# Autodesk Inventor assembly: Boost Converter
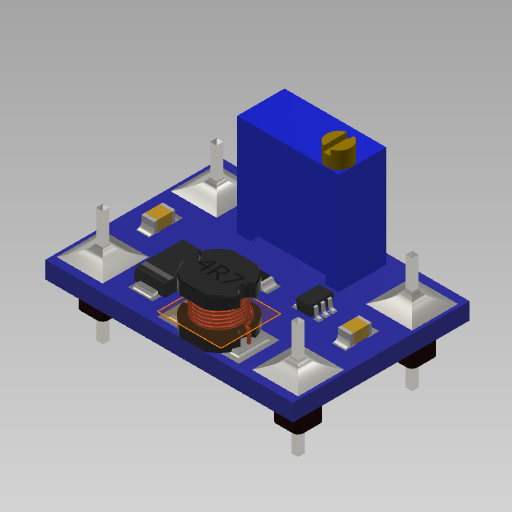
[picture p0: Inventor's stored thumbnail of the model, 512x512]
Saved by Autodesk Inventor 2020 (Build 240168000, 168)
## iProperties
Created: 2018-09-30
Part Number: Boost Converter
Document SubType Name: Weldment
Designer: amsmi
Weld Material: Titanium
Author: amsmi
## Documents named in this file (9)
- C:\Users\Alex\Google Drive\Pirani Gauge\Pirani Gauge Modeling\Data Acquisition\Boost Converter.iam
- C:\Users\Alex\Google Drive\Pirani Gauge\Pirani Gauge Modeling\Data Acquisition\Boost Converter.ipt
- C:\Users\Alex\Google Drive\Pirani Gauge\Pirani Gauge Modeling\Data Acquisition\DO-221AC.ipt
- C:\Users\Alex\Google Drive\Pirani Gauge\Pirani Gauge Modeling\Data Acquisition\Cap 0805.ipt
- C:\Users\Alex\Google Drive\Pirani Gauge\Pirani Gauge Modeling\Data Acquisition\Precision Trim Pot - baoter 3296.ipt
- C:\Users\Alex\Google Drive\Pirani Gauge\Pirani Gauge Modeling\Data Acquisition\Black 0805.ipt
- C:\Users\Alex\Google Drive\Pirani Gauge\Pirani Gauge Modeling\Data Acquisition\400nH Inductor.ipt
- C:\Users\Alex\Google Drive\Pirani Gauge\Pirani Gauge Modeling\Data Acquisition\SOT-23 6 pin.iam
- C:\Users\Alex\Google Drive\Pirani Gauge\Pirani Gauge Modeling\Data Acquisition\1 pin header.ipt
## Components (12 placed, 8 different names)
1. Boost Converter:1 — Mate:1, Mate:2, Mate:3, Mate:4, Mate:5, Mate:6, Mate:7, Angle:1, Mate:8, Angle:2, Mate:10, Angle:3, Mate:11, Flush:1, Flush:2, Flush:3, Flush:4, Flush:5, Flush:6, Flush:7, Flush:8, Mate:12, Angle:4, Flush:9, Flush:10, Mate:13, Angle:5, Flush:11, Flush:12, Mate:14, Mate:15, Mate:16
2. DO-221AC:1 — Mate:7, Angle:1, Flush:7, Flush:8
3. Cap 0805:1 — Mate:8, Angle:2, Flush:5, Flush:6
4. Cap 0805:2 — Mate:10, Angle:3, Flush:1, Flush:2
5. Black 0805:1 — Mate:11, Flush:3, Flush:4
6. Precision Trim Pot - baoter 3296:1 — Mate:1, Mate:5, Mate:6
7. 400nH Inductor:1 — Mate:12, Angle:4, Flush:9, Flush:10
8. SOT-23 6 pin:2 [sub-assembly] — Mate:13, Angle:5, Flush:11, Flush:12
9. 1 pin header:1 — Mate:14, Mate:15, Mate:16
10. 1 pin header:2
11. 1 pin header:3
12. 1 pin header:4
## Component patterns: (4 elements, first: 1 pin header:1)
## Relationships (32: Mate 15, Flush 12, Angle 5)
- Mate:1: Boost Converter:1 ↔ Precision Trim Pot - baoter 3296:1
- Mate:2: Boost Converter:1
- Mate:3: Boost Converter:1
- Mate:4: Boost Converter:1
- Mate:5: Boost Converter:1 ↔ Precision Trim Pot - baoter 3296:1
- Mate:6: Boost Converter:1 ↔ Precision Trim Pot - baoter 3296:1
- Mate:7: Boost Converter:1 ↔ DO-221AC:1
- Angle:1 (0 deg): Boost Converter:1 ↔ DO-221AC:1
- Mate:8: Boost Converter:1 ↔ Cap 0805:1
- Angle:2 (0 deg): Boost Converter:1 ↔ Cap 0805:1
- Mate:10: Boost Converter:1 ↔ Cap 0805:2
- Angle:3 (0 deg): Boost Converter:1 ↔ Cap 0805:2
- Mate:11: Boost Converter:1 ↔ Black 0805:1
- Flush:1 (7.2136 mm): Boost Converter:1 ↔ Cap 0805:2
- Flush:2 (1.8288 mm): Boost Converter:1 ↔ Cap 0805:2
- Flush:3 (10.6172 mm): Boost Converter:1 ↔ Black 0805:1
- Flush:4 (7.62 mm): Boost Converter:1 ↔ Black 0805:1
- Flush:5 (7.1628 mm): Boost Converter:1 ↔ Cap 0805:1
- Flush:6 (-1.8288 mm): Boost Converter:1 ↔ Cap 0805:1
- Flush:7 (-2.0066 mm): Boost Converter:1 ↔ DO-221AC:1
- Flush:8 (15.1384 mm): Boost Converter:1 ↔ DO-221AC:1
- Mate:12: Boost Converter:1 ↔ 400nH Inductor:1
- Angle:4 (0 deg): Boost Converter:1 ↔ 400nH Inductor:1
- Flush:9: Boost Converter:1 ↔ 400nH Inductor:1
- Flush:10 (6.35 mm): Boost Converter:1 ↔ 400nH Inductor:1
- Mate:13 (0.127 mm): Boost Converter:1 ↔ SOT-23 6 pin:2
- Angle:5 (90 deg): Boost Converter:1 ↔ SOT-23 6 pin:2
- Flush:11 (7.8486 mm): Boost Converter:1 ↔ SOT-23 6 pin:2
- Flush:12 (6.604 mm): Boost Converter:1 ↔ SOT-23 6 pin:2
- Mate:14: Boost Converter:1 ↔ 1 pin header:1
- Mate:15: Boost Converter:1 ↔ 1 pin header:1
- Mate:16: Boost Converter:1 ↔ 1 pin header:1
